# Autodesk Inventor assembly: SystemAssemV2
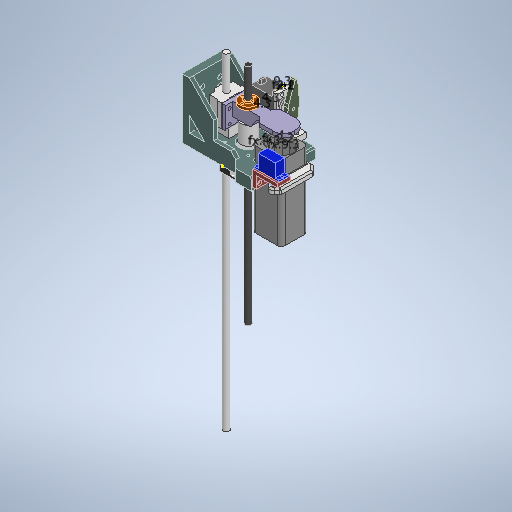
[picture p0: Inventor's stored thumbnail of the model, 512x512]
Saved by Autodesk Inventor 2025.1 (Build 291241000, 241)
## iProperties
Created: 2025-03-02
Part Number: SystemAssemV2
Document SubType Name: Assembly
Designer: 13156
Author: 13156
## Documents named in this file (18)
- C:\Users\13156\OneDrive - Binghamton University\Documents\GitHub\Perovskite-Automated-Synthesis-System\CAD\Pipette\SystemAssemV2.iam
- C:\Users\13156\OneDrive - Binghamton University\Documents\GitHub\Perovskite-Automated-Synthesis-System\CAD\Pipette\HolderV2.ipt
- C:\Users\13156\OneDrive - Binghamton University\Documents\GitHub\Perovskite-Automated-Synthesis-System\CAD\Non 3D Printed Parts\Motors and Servos\NEMA17 Stepper Motor - 26 mm.ipt
- C:\Users\13156\OneDrive - Binghamton University\Documents\GitHub\Perovskite-Automated-Synthesis-System\CAD\Pipette\Pipette Sleeve.ipt
- C:\Users\13156\OneDrive - Binghamton University\Documents\GitHub\Perovskite-Automated-Synthesis-System\CAD\Pipette\LeadScrewBase.ipt
- C:\Users\13156\OneDrive - Binghamton University\Documents\GitHub\Perovskite-Automated-Synthesis-System\CAD\Non 3D Printed Parts\Linear Rails\8mm Linear Rod.ipt
- C:\Users\13156\OneDrive - Binghamton University\Documents\GitHub\Perovskite-Automated-Synthesis-System\CAD\Non 3D Printed Parts\Linear Rails\Linear Bearing 8mm Square.ipt
- C:\Users\13156\OneDrive - Binghamton University\Documents\GitHub\Perovskite-Automated-Synthesis-System\CAD\Pipette\ActuatorV2.ipt
- C:\Users\13156\OneDrive - Binghamton University\Documents\GitHub\Perovskite-Automated-Synthesis-System\CAD\Pipette\BIGServoHolder.ipt
- C:\Users\13156\OneDrive - Binghamton University\Documents\GitHub\Perovskite-Automated-Synthesis-System\CAD\Pipette\996R.ipt
- C:\Users\13156\OneDrive - Binghamton University\Documents\GitHub\Perovskite-Automated-Synthesis-System\CAD\Non 3D Printed Parts\Leadscrew.ipt
- C:\Users\13156\OneDrive - Binghamton University\Documents\GitHub\Perovskite-Automated-Synthesis-System\CAD\Pipette\BigServoEjectorArm.ipt
- C:\Users\13156\OneDrive - Binghamton University\Documents\GitHub\Perovskite-Automated-Synthesis-System\CAD\Non 3D Printed Parts\Threaded Rod 300mm.ipt
- C:\Users\13156\OneDrive - Binghamton University\Documents\GitHub\Perovskite-Automated-Synthesis-System\CAD\Pipette\GrabberServoHolder.ipt
- C:\Users\13156\OneDrive - Binghamton University\Documents\GitHub\Perovskite-Automated-Synthesis-System\CAD\Non 3D Printed Parts\Motors and Servos\SG90 Servo.ipt
- C:\Users\13156\OneDrive - Binghamton University\Documents\GitHub\Perovskite-Automated-Synthesis-System\CAD\Pipette\GrabberArmV2.ipt
- C:\Users\13156\OneDrive - Binghamton University\Documents\GitHub\Perovskite-Automated-Synthesis-System\CAD\Pipette\HalfServoArm.ipt
- C:\Users\13156\OneDrive - Binghamton University\Documents\GitHub\Perovskite-Automated-Synthesis-System\CAD\Non 3D Printed Parts\Linear Rails\Linear Rod Holder SK8.ipt
## Components (17 placed, 17 different names)
1. HolderV2:1 — Mate:1, Mate:2, Mate:3, Mate:4, Mate:5, Mate:6, Mate:7, Mate:8, Mate:9, Mate:10, Mate:13, Mate:19, Mate:20, Mate:21, Mate:26, Mate:27, Mate:28, Flush:1, Flush:3, Mate:42, Mate:43, Mate:44, Mate:52, Mate:53, Mate:54
2. NEMA17 Stepper Motor - 26 mm:1 — Mate:4, Mate:5, Mate:6, Mate:7, Mate:11, Mate:41
3. Pipette Sleeve:1 — Mate:8, Mate:9, Mate:10
4. LeadScrewBase:1 — Mate:11, Mate:28, Mate:30, Mate:40
5. 8mm Linear Rod:1 — Mate:13, Mate:14, Flush:1, Flush:2
6. Linear Bearing 8mm Square:1 — Mate:14, Mate:16, Mate:29
7. ActuatorV2:1 — Mate:16, Mate:29, Mate:30, Mate:31, Mate:32, Mate:33, Mate:34
8. BIGServoHolder:1 — Mate:19, Mate:20, Mate:21, Mate:24, Mate:26, Mate:27, Mate:36, Mate:37
9. 996R:1 — Mate:24, Mate:36, Mate:37, Mate:38, Mate:39
10. Leadscrew:1 — Mate:31, Mate:32, Mate:33, Mate:34, Mate:40
11. BigServoEjectorArm:1 — Mate:38, Mate:39
12. Threaded Rod 300mm:1 — Mate:41, Flush:2, Flush:3
13. GrabberServoHolder:1 — Mate:42, Mate:43, Mate:44, Mate:45, Mate:46, Mate:47
14. SG90 Servo:1 — Mate:45, Mate:46, Mate:47, Mate:48, Mate:49
15. GrabberArmV2:1 — Mate:50, Mate:51
16. HalfServoArm:1 — Mate:48, Mate:49, Mate:50, Mate:51
17. Linear Rod Holder SK8:1 — Mate:52, Mate:53, Mate:54
## Relationships (49: Mate 46, Flush 3)
- Mate:1: HolderV2:1
- Mate:2: HolderV2:1
- Mate:3: HolderV2:1
- Mate:4: HolderV2:1 ↔ NEMA17 Stepper Motor - 26 mm:1
- Mate:5: HolderV2:1 ↔ NEMA17 Stepper Motor - 26 mm:1
- Mate:6: HolderV2:1 ↔ NEMA17 Stepper Motor - 26 mm:1
- Mate:7: HolderV2:1 ↔ NEMA17 Stepper Motor - 26 mm:1
- Mate:8: HolderV2:1 ↔ Pipette Sleeve:1
- Mate:9: HolderV2:1 ↔ Pipette Sleeve:1
- Mate:10: HolderV2:1 ↔ Pipette Sleeve:1
- Mate:11: NEMA17 Stepper Motor - 26 mm:1 ↔ LeadScrewBase:1
- Mate:13: HolderV2:1 ↔ 8mm Linear Rod:1
- Mate:14: 8mm Linear Rod:1 ↔ Linear Bearing 8mm Square:1
- Mate:16: Linear Bearing 8mm Square:1 ↔ ActuatorV2:1
- Mate:19: HolderV2:1 ↔ BIGServoHolder:1
- Mate:20: HolderV2:1 ↔ BIGServoHolder:1
- Mate:21: HolderV2:1 ↔ BIGServoHolder:1
- Mate:24: BIGServoHolder:1 ↔ 996R:1
- Mate:26: HolderV2:1 ↔ BIGServoHolder:1
- Mate:27: HolderV2:1 ↔ BIGServoHolder:1
- Mate:28 (2 mm): HolderV2:1 ↔ LeadScrewBase:1
- Flush:1 (-90 mm): HolderV2:1 ↔ 8mm Linear Rod:1
- Mate:29: Linear Bearing 8mm Square:1 ↔ ActuatorV2:1
- Mate:30: LeadScrewBase:1 ↔ ActuatorV2:1
- Mate:31: ActuatorV2:1 ↔ Leadscrew:1
- Mate:32: ActuatorV2:1 ↔ Leadscrew:1
- Mate:33: ActuatorV2:1 ↔ Leadscrew:1
- Mate:34: ActuatorV2:1 ↔ Leadscrew:1
- Mate:36: BIGServoHolder:1 ↔ 996R:1
- Mate:37 (0.5 mm): BIGServoHolder:1 ↔ 996R:1
- Mate:38: 996R:1 ↔ BigServoEjectorArm:1
- Mate:39: 996R:1 ↔ BigServoEjectorArm:1
- Mate:40: LeadScrewBase:1 ↔ Leadscrew:1
- Mate:41: NEMA17 Stepper Motor - 26 mm:1 ↔ Threaded Rod 300mm:1
- Flush:2: 8mm Linear Rod:1 ↔ Threaded Rod 300mm:1
- Flush:3 (-90 mm): HolderV2:1 ↔ Threaded Rod 300mm:1
- Mate:42: HolderV2:1 ↔ GrabberServoHolder:1
- Mate:43: HolderV2:1 ↔ GrabberServoHolder:1
- Mate:44: HolderV2:1 ↔ GrabberServoHolder:1
- Mate:45: GrabberServoHolder:1 ↔ SG90 Servo:1
- Mate:46: GrabberServoHolder:1 ↔ SG90 Servo:1
- Mate:47: GrabberServoHolder:1 ↔ SG90 Servo:1
- Mate:48: SG90 Servo:1 ↔ HalfServoArm:1
- Mate:49 (1 mm): SG90 Servo:1 ↔ HalfServoArm:1
- Mate:50: GrabberArmV2:1 ↔ HalfServoArm:1
- Mate:51: GrabberArmV2:1 ↔ HalfServoArm:1
- Mate:52: HolderV2:1 ↔ Linear Rod Holder SK8:1
- Mate:53: HolderV2:1 ↔ Linear Rod Holder SK8:1
- Mate:54: HolderV2:1 ↔ Linear Rod Holder SK8:1
